# Autodesk Inventor assembly: SKF_SY 7/8 TF
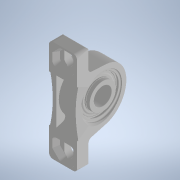
[picture p0: Inventor's stored thumbnail of the model, 180x180]
Saved by Autodesk Inventor 2021 (Build 250183000, 183)
## iProperties
Category: PARTsolutions
Company: SKF
Created: 2025-11-05
Part Number: SKF_SY 7/8 TF
Catalog Web Link: www.3dfindit.com
Description: AYP_001_HC_HH_HY-AYL_001_HP-Y-bearing plummer block units
Vendor: SKF
Document SubType Name: Assembly
Designer: psAdmin
Manufacturer: SKF
Mass: 296.697 g
Surface Area: 494.643 cm^2
Volume: 102.457 cm^3
Density: 2.8958 g/cm^3
Title: SKF_SY 7/8 TF
Author: Cadenas PARTsolutions
Comments: Y-bearing plummer block units
PSOL_IDENT_0: {$CADENAS_DATA/23d-libs/skf/bearings_units_and_housings/bearing_units/ball_bearing_units/y-units/ayp
PSOL_IDENT_1: _001_hc_hh_hy-ayl_001_hp.prj},208 {VTYP=3D},{STYP=ASSTAB},{NB=SKF_SY 7/8 TF},{LINA=SKF_SY 7/8 TF},{N
PSOL_IDENT_2: N=AYP_001_HC_HH_HY-AYL_001_HP},{DATE=03.11.2025 06:54:15},{GEOMDATE=09.09.2025 06:52:47},{VERSION=},
PSOL_IDENT_3: {LINEID=4710},{WBVAR=COVER},{WBNUMERIC=}  {NB=SKF_SY 7/8 TF},{LINA=SKF_SY 7/8 TF},{KT=DUMMY},{DESIGN
PSOL_IDENT_4: ATION=SY 7/8 TF},{COVER=},{DDALG=22.2250},{DD=22.225},{DDX=},{DD1=33.74},{DD2=},{DAA=},{HA=},{A=36.0
PSOL_IDENT_5: 00},{AX=},{AXX=},{AXXX=},{A1=22.000},{A1X=},{A1XX=},{A1XXX=},{A5=20.500},{A5X=},{A5XX=},{B=34.100},{
PSOL_IDENT_6: B1=34.100},{B1X=},{B4ALG=5.000},{B4=5},{B4X=},{H=70},{HX=},{HXX=},{HXXX=},{H1=36.5},{H1X=},{H1XX=},{
PSOL_IDENT_7: H1XXX=},{H2=16},{H2X=},{H2XX=},{H2XXX=},{J=102},{JX=},{JXX=},{JXXX=},{JMAX=110},{JMAXX=},{JMAXXX=},{
PSOL_IDENT_8: JMIN=94},{JMINX=},{JMINXX=},{L=130},{LX=},{LXX=},{LXXX=},{N=19.5},{NX=},{NXX=},{NXXX=},{N1=11.5},{N1
PSOL_IDENT_9: X=},{N1XX=},{N1XXX=},{SS1=19.8},{SS1X=19.8},{RG=1/4-28 UNF},{RGX=},{R1=2},{R1X=},{RALPHA=45.00000000
PSOL_IDENT_10: 0112},{RALPHAX=},{DN=6.5},{SWN=7},{GN=1/4-28 SAE-LT},{J6=120},{J7=13},{D=52},{D1=52},{C=15},{R12=0.6
PSOL_IDENT_11: },{B3=},{DW=7.938},{PITCH=39.040},{LOAD1=14},{LOAD2=7.8},{LOAD3=0.335},{SPEED1=7000},{II=1},{Z=9},{M
PSOL_IDENT_12: ASS=0.75},{MASSX=},{MASSXX=},{G2=1/4-28 UNF},{HKSGS=3.175},{RTTGS=4},{AS=},{ALPHA=},{G=10},{GX=},{GX
PSOL_IDENT_13: X=},{GXXX=},{GIN=0.375000002475},{GINX=},{GINXX=},{GINXXX=},{HOUSING=SY 505 M},{HOUSINGX=},{HOUSINGX
PSOL_IDENT_14: X=},{HOUSINGXXX=},{BEARING=YAR 205-014-2F},{BEARINGX=},{SLEEVE=},{BS=},{RING=},{ECALG=ECY 205},{EC=}
PSOL_IDENT_15: ,{ECX=ECY 205},{ECXX=},{ECXXX=},{POPULAR=},{PPATH=y-bearing_plummer_block_units_parts/ayp_001_hc_hh_
PSOL_IDENT_16: hy-ayl_001_hp_asmtpl.prj},{COVERALG=  '', 'No end cover', 'ECY 205', 'ECY 205' },{SUPPRESSED=0},{DES
PSOL_IDENT_17: IGN=sy},{TC=SY 7/8 TF},{COVERX=0}
NB: SKF_SY 7/8 TF
NN: AYP_001_HC_HH_HY-AYL_001_HP
NT: Y-bearing plummer block units
NBSYN: SKF_$TC.
LINA: SKF_SY 7/8 TF
CATALOG: SKF
DESIGNATION: SY 7/8 TF
COVER: No end cover
DDALG: 22.225
DD1: 33.74
A: 36
A1: 22
A5: 20.5
B: 34.1
B1: 34.1
B4ALG: 5
H: 70
H1: 36.5
H2: 16
J: 102
JMAX: 110
JMIN: 94
L: 130
N: 19.5
N1: 11.5
SS1: 19.8
RG: 1/4-28 UNF
R1: 2
RALPHA: 45.000000000112
DN: 6.5
SWN: 7
GN: 1/4-28 SAE-LT
J6: 120
J7: 13
LOAD1: 14
LOAD2: 7.8
LOAD3: 0.335
SPEED1: 7000
MASS: 0.75
G2: 1/4-28 UNF
HKSGS: 3.175
RTTGS: 4
G: 10
GIN: 0.375000002475
HOUSING: SY 505 M
BEARING: YAR 205-014-2F
COVERX: 0
SUPPLIER: SKF
ARTICLENO: SKF_SY 7/8 TF
BOMINFO: SKF_SY 7/8 TF
CREATOR: CADENAS GmbH
## Documents named in this file (5)
- e:\temp\worker_COMMON_2\temp\tmp_9040_26_ZltIq\format_0\SKF_SY 7_8 TF.iam
- e:\temp\worker_COMMON_2\temp\tmp_9040_26_ZltIq\format_0\housingSY 505 M-h.ipt
- e:\temp\worker_COMMON_2\temp\tmp_9040_26_ZltIq\format_0\1_4-28 SAE-LT.ipt
- e:\temp\worker_COMMON_2\temp\tmp_9040_26_ZltIq\format_0\YAR 205-014-2F-33_740-b.ipt
- e:\temp\worker_COMMON_2\temp\tmp_9040_26_ZltIq\format_0\22_225-52-34_1-15-ybrg1-507_938-39_04-b.ipt
## Components (12 placed, 4 different names)
1. housingSY 505 M-h:1 — gn_1_XY@1 <-> gn_XY@2, gn_1_Z@1 <-> gn_Z@2, gn_1_YZ@1 <-> gn_YZ@2
2. 1_4-28 SAE-LT:1 — gn_1_XY@1 <-> gn_XY@2, gn_1_Z@1 <-> gn_Z@2, gn_1_YZ@1 <-> gn_YZ@2
3. YAR 205-014-2F-33_740-b:1 — ball_1_XY@3 <-> ball_XY@4, ball_1_Z@3 <-> ball_Z@4, ball_1_YZ@3 <-> ball_YZ@4, ball_2_XY@3 <-> ball_XY@5, ball_2_Z@3 <-> ball_Z@5, ball_2_YZ@3 <-> ball_YZ@5, ball_3_XY@3 <-> ball_XY@6, ball_3_Z@3 <-> ball_Z@6, ball_3_YZ@3 <-> ball_YZ@6, ball_4_XY@3 <-> ball_XY@7, ball_4_Z@3 <-> ball_Z@7, ball_4_YZ@3 <-> ball_YZ@7, ball_5_XY@3 <-> ball_XY@8, ball_5_Z@3 <-> ball_Z@8, ball_5_YZ@3 <-> ball_YZ@8, ball_6_XY@3 <-> ball_XY@9, ball_6_Z@3 <-> ball_Z@9, ball_6_YZ@3 <-> ball_YZ@9, ball_7_XY@3 <-> ball_XY@10, ball_7_Z@3 <-> ball_Z@10, ball_7_YZ@3 <-> ball_YZ@10, ball_8_XY@3 <-> ball_XY@11, ball_8_Z@3 <-> ball_Z@11, ball_8_YZ@3 <-> ball_YZ@11, ball_9_XY@3 <-> ball_XY@12, ball_9_Z@3 <-> ball_Z@12, ball_9_YZ@3 <-> ball_YZ@12
4. 22_225-52-34_1-15-ybrg1-507_938-39_04-b:1 — ball_1_XY@3 <-> ball_XY@4, ball_1_Z@3 <-> ball_Z@4, ball_1_YZ@3 <-> ball_YZ@4
5. 22_225-52-34_1-15-ybrg1-507_938-39_04-b:2 — ball_2_XY@3 <-> ball_XY@5, ball_2_Z@3 <-> ball_Z@5, ball_2_YZ@3 <-> ball_YZ@5
6. 22_225-52-34_1-15-ybrg1-507_938-39_04-b:3 — ball_3_XY@3 <-> ball_XY@6, ball_3_Z@3 <-> ball_Z@6, ball_3_YZ@3 <-> ball_YZ@6
7. 22_225-52-34_1-15-ybrg1-507_938-39_04-b:4 — ball_4_XY@3 <-> ball_XY@7, ball_4_Z@3 <-> ball_Z@7, ball_4_YZ@3 <-> ball_YZ@7
8. 22_225-52-34_1-15-ybrg1-507_938-39_04-b:5 — ball_5_XY@3 <-> ball_XY@8, ball_5_Z@3 <-> ball_Z@8, ball_5_YZ@3 <-> ball_YZ@8
9. 22_225-52-34_1-15-ybrg1-507_938-39_04-b:6 — ball_6_XY@3 <-> ball_XY@9, ball_6_Z@3 <-> ball_Z@9, ball_6_YZ@3 <-> ball_YZ@9
10. 22_225-52-34_1-15-ybrg1-507_938-39_04-b:7 — ball_7_XY@3 <-> ball_XY@10, ball_7_Z@3 <-> ball_Z@10, ball_7_YZ@3 <-> ball_YZ@10
11. 22_225-52-34_1-15-ybrg1-507_938-39_04-b:8 — ball_8_XY@3 <-> ball_XY@11, ball_8_Z@3 <-> ball_Z@11, ball_8_YZ@3 <-> ball_YZ@11
12. 22_225-52-34_1-15-ybrg1-507_938-39_04-b:9 — ball_9_XY@3 <-> ball_XY@12, ball_9_Z@3 <-> ball_Z@12, ball_9_YZ@3 <-> ball_YZ@12
## Relationships (30: Mate 19, Angle 10, Flush 1)
- gn_1_XY@1 <-> gn_XY@2 [Flush]: housingSY 505 M-h:1 ↔ 1_4-28 SAE-LT:1
- gn_1_Z@1 <-> gn_Z@2 [Mate]: housingSY 505 M-h:1 ↔ 1_4-28 SAE-LT:1
- gn_1_YZ@1 <-> gn_YZ@2 [Angle] (0 deg): housingSY 505 M-h:1 ↔ 1_4-28 SAE-LT:1
- ball_1_XY@3 <-> ball_XY@4 [Mate]: YAR 205-014-2F-33_740-b:1 ↔ 22_225-52-34_1-15-ybrg1-507_938-39_04-b:1
- ball_1_Z@3 <-> ball_Z@4 [Mate]: YAR 205-014-2F-33_740-b:1 ↔ 22_225-52-34_1-15-ybrg1-507_938-39_04-b:1
- ball_1_YZ@3 <-> ball_YZ@4 [Angle] (0 deg): YAR 205-014-2F-33_740-b:1 ↔ 22_225-52-34_1-15-ybrg1-507_938-39_04-b:1
- ball_2_XY@3 <-> ball_XY@5 [Mate]: YAR 205-014-2F-33_740-b:1 ↔ 22_225-52-34_1-15-ybrg1-507_938-39_04-b:2
- ball_2_Z@3 <-> ball_Z@5 [Mate]: YAR 205-014-2F-33_740-b:1 ↔ 22_225-52-34_1-15-ybrg1-507_938-39_04-b:2
- ball_2_YZ@3 <-> ball_YZ@5 [Angle] (0 deg): YAR 205-014-2F-33_740-b:1 ↔ 22_225-52-34_1-15-ybrg1-507_938-39_04-b:2
- ball_3_XY@3 <-> ball_XY@6 [Mate]: YAR 205-014-2F-33_740-b:1 ↔ 22_225-52-34_1-15-ybrg1-507_938-39_04-b:3
- ball_3_Z@3 <-> ball_Z@6 [Mate]: YAR 205-014-2F-33_740-b:1 ↔ 22_225-52-34_1-15-ybrg1-507_938-39_04-b:3
- ball_3_YZ@3 <-> ball_YZ@6 [Angle] (0 deg): YAR 205-014-2F-33_740-b:1 ↔ 22_225-52-34_1-15-ybrg1-507_938-39_04-b:3
- ball_4_XY@3 <-> ball_XY@7 [Mate]: YAR 205-014-2F-33_740-b:1 ↔ 22_225-52-34_1-15-ybrg1-507_938-39_04-b:4
- ball_4_Z@3 <-> ball_Z@7 [Mate]: YAR 205-014-2F-33_740-b:1 ↔ 22_225-52-34_1-15-ybrg1-507_938-39_04-b:4
- ball_4_YZ@3 <-> ball_YZ@7 [Angle] (0 deg): YAR 205-014-2F-33_740-b:1 ↔ 22_225-52-34_1-15-ybrg1-507_938-39_04-b:4
- ball_5_XY@3 <-> ball_XY@8 [Mate]: YAR 205-014-2F-33_740-b:1 ↔ 22_225-52-34_1-15-ybrg1-507_938-39_04-b:5
- ball_5_Z@3 <-> ball_Z@8 [Mate]: YAR 205-014-2F-33_740-b:1 ↔ 22_225-52-34_1-15-ybrg1-507_938-39_04-b:5
- ball_5_YZ@3 <-> ball_YZ@8 [Angle] (0 deg): YAR 205-014-2F-33_740-b:1 ↔ 22_225-52-34_1-15-ybrg1-507_938-39_04-b:5
- ball_6_XY@3 <-> ball_XY@9 [Mate]: YAR 205-014-2F-33_740-b:1 ↔ 22_225-52-34_1-15-ybrg1-507_938-39_04-b:6
- ball_6_Z@3 <-> ball_Z@9 [Mate]: YAR 205-014-2F-33_740-b:1 ↔ 22_225-52-34_1-15-ybrg1-507_938-39_04-b:6
- ball_6_YZ@3 <-> ball_YZ@9 [Angle] (0 deg): YAR 205-014-2F-33_740-b:1 ↔ 22_225-52-34_1-15-ybrg1-507_938-39_04-b:6
- ball_7_XY@3 <-> ball_XY@10 [Mate]: YAR 205-014-2F-33_740-b:1 ↔ 22_225-52-34_1-15-ybrg1-507_938-39_04-b:7
- ball_7_Z@3 <-> ball_Z@10 [Mate]: YAR 205-014-2F-33_740-b:1 ↔ 22_225-52-34_1-15-ybrg1-507_938-39_04-b:7
- ball_7_YZ@3 <-> ball_YZ@10 [Angle] (0 deg): YAR 205-014-2F-33_740-b:1 ↔ 22_225-52-34_1-15-ybrg1-507_938-39_04-b:7
- ball_8_XY@3 <-> ball_XY@11 [Mate]: YAR 205-014-2F-33_740-b:1 ↔ 22_225-52-34_1-15-ybrg1-507_938-39_04-b:8
- ball_8_Z@3 <-> ball_Z@11 [Mate]: YAR 205-014-2F-33_740-b:1 ↔ 22_225-52-34_1-15-ybrg1-507_938-39_04-b:8
- ball_8_YZ@3 <-> ball_YZ@11 [Angle] (0 deg): YAR 205-014-2F-33_740-b:1 ↔ 22_225-52-34_1-15-ybrg1-507_938-39_04-b:8
- ball_9_XY@3 <-> ball_XY@12 [Mate]: YAR 205-014-2F-33_740-b:1 ↔ 22_225-52-34_1-15-ybrg1-507_938-39_04-b:9
- ball_9_Z@3 <-> ball_Z@12 [Mate]: YAR 205-014-2F-33_740-b:1 ↔ 22_225-52-34_1-15-ybrg1-507_938-39_04-b:9
- ball_9_YZ@3 <-> ball_YZ@12 [Angle] (0 deg): YAR 205-014-2F-33_740-b:1 ↔ 22_225-52-34_1-15-ybrg1-507_938-39_04-b:9
